# Autodesk Inventor assembly: Chestbox_with_electronical_devices
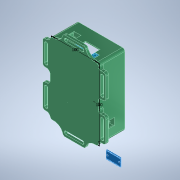
[picture p0: Inventor's stored thumbnail of the model, 180x180]
Saved by Autodesk Inventor 2021 (Build 250183000, 183)
## iProperties
Created: 2021-12-04
Part Number: Chestbox_with_electronical_devices
Document SubType Name: Assembly
Designer: marcin
Author: marcin
## Documents named in this file (8)
- C:\Users\marcin\Desktop\Motion_capture\MAIN\Models_3D\Chest_box\Chestbox_with_electronical_devices.iam
- C:\Users\marcin\Desktop\Motion_capture\MAIN\Models_3D\Chest_box\chestbox.ipt
- C:\Users\marcin\Desktop\Motion_capture\MAIN\Models_3D\Chest_box\ArduinoMega_STEP_AP203.ipt
- C:\Users\marcin\Desktop\Motion_capture\MAIN\Models_3D\Chest_box\TCA9548A Adfruit with Header.iam
- C:\Users\marcin\Desktop\Motion_capture\MAIN\Models_3D\Chest_box\BNO055_Xplained_pro(Default_assembly).iam
- C:\Users\marcin\Desktop\Motion_capture\MAIN\Models_3D\Chest_box\do druku\lid.ipt
- C:\Users\marcin\Desktop\Motion_capture\MAIN\Models_3D\Chest_box\STEP 1602 Serial LCD Module.ipt
- C:\Users\marcin\Desktop\Tefal-koło\modelkoła\Design Accelerator\arduino_fastening.ipt
## Components (7 placed, 7 different names)
1. chestbox:1 — Mate:1, Flush:1, Mate:2, Mate:3, Mate:4, Mate:5, Mate:9, Mate:10, Mate:11, Flush:2, Flush:15
2. ArduinoMega_STEP_AP203:1 — Mate:3, Mate:4, Mate:5
3. TCA9548A Adfruit with Header:1 [sub-assembly]
4. BNO055_Xplained_pro(Default_assembly):1 [sub-assembly] — Mate:9, Mate:10, Mate:11
5. lid:1 — Flush:2, Flush:13, Mate:13
6. STEP 1602 Serial LCD Module:1 — Flush:13, Mate:13, Flush:14
7. arduino_fastening:1 — Flush:15
## Relationships (14: Mate 9, Flush 5)
- Mate:1: chestbox:1
- Flush:1: chestbox:1
- Mate:2: chestbox:1
- Mate:3: chestbox:1 ↔ ArduinoMega_STEP_AP203:1
- Mate:4: chestbox:1 ↔ ArduinoMega_STEP_AP203:1
- Mate:5 (10 mm): chestbox:1 ↔ ArduinoMega_STEP_AP203:1
- Mate:9: chestbox:1 ↔ BNO055_Xplained_pro(Default_assembly):1
- Mate:10: chestbox:1 ↔ BNO055_Xplained_pro(Default_assembly):1
- Mate:11: chestbox:1 ↔ BNO055_Xplained_pro(Default_assembly):1
- Flush:2: chestbox:1 ↔ lid:1
- Flush:13: lid:1 ↔ STEP 1602 Serial LCD Module:1
- Mate:13: lid:1 ↔ STEP 1602 Serial LCD Module:1
- Flush:14: STEP 1602 Serial LCD Module:1
- Flush:15: chestbox:1 ↔ arduino_fastening:1
